# Autodesk Inventor assembly: Assembly1
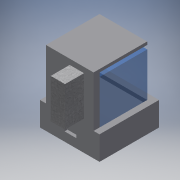
[picture p0: Inventor's stored thumbnail of the model, 180x180]
Saved by Autodesk Inventor 2016 (Build 200138000, 138)
## iProperties
Created: 2016-08-06
Part Number: Assembly1
Document SubType Name: Assembly
Designer: Jorian Brusind
Author: Jorian Brusind
## Documents named in this file (4)
- C:\Users\Jorian Brusind\Desktop\Auto Terrarium\Assembly1.iam
- C:\Users\Jorian Brusind\Desktop\Auto Terrarium\Part2.ipt
- C:\Users\Jorian Brusind\Desktop\Auto Terrarium\Motor.ipt
- C:\Users\Jorian Brusind\Desktop\Auto Terrarium\model for case.ipt
## Components (3 placed, 3 different names)
1. Part2:1 — Mate:1, Mate:2, Mate:3
2. Motor:1 — Mate:4, Flush:1, Flush:2
3. model for case:1 — Mate:1, Mate:2, Mate:3, Mate:4, Flush:1, Flush:2
## Relationships (6: Mate 4, Flush 2)
- Mate:1: Part2:1 ↔ model for case:1
- Mate:2: Part2:1 ↔ model for case:1
- Mate:3: Part2:1 ↔ model for case:1
- Mate:4: Motor:1 ↔ model for case:1
- Flush:1 (63.5 mm): Motor:1 ↔ model for case:1
- Flush:2 (-63.5 mm): Motor:1 ↔ model for case:1
